# Autodesk Inventor assembly: Assembly_Cube_SEEED_Xiao_Sense_Camera_adapter_v3
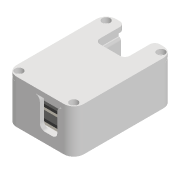
[picture p0: Inventor's stored thumbnail of the model, 180x180]
Saved by Autodesk Inventor 2022 (Build 260153000, 153)
## iProperties
Created: 2023-04-26
Part Number: Assembly_Cube_SEEED_Xiao_Sense_Camera_adapter_v3
Document SubType Name: Assembly
Designer: diederichbenedict
Author: diederichbenedict
## Documents named in this file (6)
- C:\Users\diederichbenedict\Dropbox\Dokumente\Promotion\PROJECTS\openUC2-CAD\INVENTOR\Assembly_Cube_SEEED_Xiao_Sense_Camera_adapter_v3.iam
- C:\Users\diederichbenedict\Dropbox\Dokumente\Promotion\PROJECTS\openUC2-CAD\INVENTOR\00_Seeeduino Xiao.ipt
- C:\Users\diederichbenedict\Dropbox\Dokumente\Promotion\PROJECTS\openUC2-CAD\INVENTOR\00_ESP3-CAM.ipt
- C:\Users\diederichbenedict\Dropbox\Dokumente\Promotion\PROJECTS\openUC2-CAD\INVENTOR\00_ESP32_XIAO_Adapter_base.ipt
- C:\Users\diederichbenedict\Dropbox\Dokumente\Promotion\PROJECTS\openUC2-CAD\INVENTOR\00_ESP32_XIAO_Adapter_lid.ipt
- C:\Users\diederichbenedict\Dropbox\Dokumente\Promotion\PROJECTS\openUC2-CAD\INVENTOR\00_ESP32_XIAO_Adapter_SDcard.ipt
## Components (5 placed, 5 different names)
1. 00_Seeeduino Xiao:1 — Passend:1, Winkel:1, Fluchtend:3
2. 00_ESP32_XIAO_Adapter_base:1 — Fluchtend:1, Passend:2, Fluchtend:2, Winkel:1, Fluchtend:3, Einfügen:1, Fluchtend:4, Fluchtend:5, Passend:3
3. 00_ESP3-CAM:1 — Einfügen:1, Winkel:2
4. 00_ESP32_XIAO_Adapter_lid:1 — Fluchtend:4, Fluchtend:5, Passend:3
5. 00_ESP32_XIAO_Adapter_SDcard:1
## Relationships (11: Flush 5, Mate 3, Angle 2, Insert 1)
- Passend:1 [Mate]: 00_Seeeduino Xiao:1
- Fluchtend:1 [Flush]: 00_ESP32_XIAO_Adapter_base:1
- Passend:2 [Mate]: 00_ESP32_XIAO_Adapter_base:1
- Fluchtend:2 [Flush]: 00_ESP32_XIAO_Adapter_base:1
- Winkel:1 [Angle] (180 deg): 00_Seeeduino Xiao:1 ↔ 00_ESP32_XIAO_Adapter_base:1
- Fluchtend:3 [Flush] (5 mm): 00_Seeeduino Xiao:1 ↔ 00_ESP32_XIAO_Adapter_base:1
- Einfügen:1 [Insert] (2.3 mm): 00_ESP32_XIAO_Adapter_base:1 ↔ 00_ESP3-CAM:1
- Winkel:2 [Angle] (180 deg): 00_ESP3-CAM:1
- Fluchtend:4 [Flush]: 00_ESP32_XIAO_Adapter_base:1 ↔ 00_ESP32_XIAO_Adapter_lid:1
- Fluchtend:5 [Flush]: 00_ESP32_XIAO_Adapter_base:1 ↔ 00_ESP32_XIAO_Adapter_lid:1
- Passend:3 [Mate]: 00_ESP32_XIAO_Adapter_base:1 ↔ 00_ESP32_XIAO_Adapter_lid:1
